# Autodesk Inventor assembly: xzrailassembly
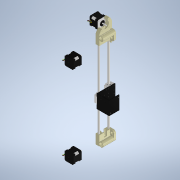
[picture p0: Inventor's stored thumbnail of the model, 180x180]
Saved by Autodesk Inventor 2020.2 (Build 242310000, 310)
## iProperties
Created: 2020-07-30
Part Number: xzrailassembly
Document SubType Name: Assembly
Designer: JK
Author: JK
## Documents named in this file (3)
- C:\Users\JK\Documents\Inventor\Anet Upgrade\xzrailassembly.iam
- C:\Users\JK\Documents\Inventor\Anet Upgrade\MOTOR.ipt
- C:\Users\JK\Documents\Inventor\Anet Upgrade\assemblyxrail.iam
## Components (3 placed, 2 different names)
1. MOTOR:2 — Flush:3, Flush:4
2. MOTOR:3 — Flush:3, Flush:4
3. assemblyxrail:1 [sub-assembly]
## Relationships (5: Flush 2, Mate 2, Angle 1)
- Flush:3: MOTOR:2 ↔ MOTOR:3
- [Mate]: MOTOR:2 ↔ assemblyxrail:1
- [Mate]: MOTOR:3 ↔ assemblyxrail:1
- [Angle] (0 deg): MOTOR:3 ↔ assemblyxrail:1
- Flush:4: MOTOR:2 ↔ MOTOR:3
